# Autodesk Inventor assembly: ASY NDM-VOS_powder_hopper
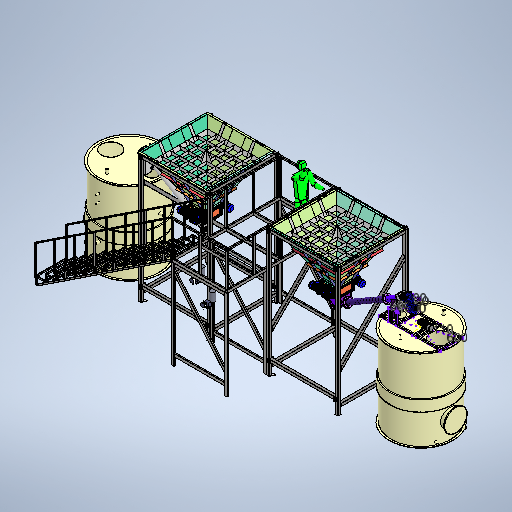
[picture p0: Inventor's stored thumbnail of the model, 512x512]
Saved by Autodesk Inventor 2025 (Build 290162010, 162A)
## iProperties
Created: 2024-07-24
Part Number: ASY NDM-VOS_powder_hopper
Document SubType Name: Assembly
Designer: admin
Author: admin
## Documents named in this file (28)
- C:\Users\pokla\Documents\Inventor\NDM-VOS_powder_hopper\ASY NDM-VOS_powder_hopper.iam
- C:\Users\pokla\Documents\Inventor\NDM-VOS_powder_hopper\human 01\ч ASY human dummy 01.iam
- C:\Users\pokla\Documents\Inventor\NDM-VOS_powder_hopper\NDM-VOS dummy3.ipt
- C:\Users\pokla\Documents\Inventor\NDM-VOS_powder_hopper\NDM-VOS dummy FLOOR.ipt
- C:\Users\pokla\Documents\Inventor\NDM-VOS_powder_hopper\NDM-VOS dummy Crane.ipt
- C:\Users\pokla\Documents\Inventor\NDM-VOS_powder_hopper\NDM-VOS dummy upstairse.ipt
- C:\Users\pokla\Documents\Inventor\NDM-VOS_powder_hopper\Workspaces\Workspace\Cone\ASY MSC 100 cone.iam
- C:\Users\pokla\Documents\Inventor\NDM-VOS_powder_hopper\ASY HPR 200  Frame.iam
- C:\Users\pokla\Documents\Inventor\NDM-VOS_powder_hopper\TM06198C pump.ipt
- C:\Users\pokla\Documents\Inventor\NDM-VOS_powder_hopper\ASY_Ступень.iam
- C:\Users\pokla\Documents\Inventor\NDM-VOS_powder_hopper\ASY стойка.iam
- C:\Users\pokla\Documents\Inventor\NDM-VOS_powder_hopper\ASY NVPH-400 shredder.iam
- C:\Users\admin\YandexDisk-badmisterfox\домашниий пк\Inventor\Content Center Files\en-US\ISO 4775\ISO 4775 - M12.ipt
- C:\Users\pokla\Documents\Inventor\NDM-VOS_powder_hopper\ASY NVPH-300 hopper.iam
- C:\Users\pokla\Documents\Inventor\NDM-VOS_powder_hopper\ASY Augur motor frame 500.iam
- C:\Users\pokla\Documents\Inventor\NDM-VOS_powder_hopper\3d party\motor-reductor NMRV040\motor-reductor NMRV040.iam
- C:\Users\pokla\Documents\Inventor\NDM-VOS_powder_hopper\3d party\Mixer 22.04.24\ASY mixer 3.iam
- C:\Users\pokla\Documents\Inventor\NDM-VOS_powder_hopper\NDM-VOS 777 sredder wall 7.ipt
- C:\Users\pokla\Documents\Inventor\NDM-VOS_powder_hopper\NDM-VOS 778 engine plate.ipt
- C:\Users\pokla\Documents\Inventor\NDM-VOS_powder_hopper\3d party\PCRV071-063SHFA_MS71B5\PCRV071-063SHFA_MS71B5\PCRV071-063SHFA_MS71B5.ipt
- C:\Users\pokla\Documents\Inventor\NDM-VOS_powder_hopper\NDM-VOS 712 flange.ipt
- C:\Users\pokla\Documents\Inventor\NDM-VOS_powder_hopper\NDM-VOS 913 flange bolt.ipt
- C:\Users\pokla\Documents\Inventor\NDM-VOS_powder_hopper\NDM-VOS 715 flange.ipt
- C:\Users\pokla\Documents\Inventor\NDM-VOS_powder_hopper\FL3.6.2  Motor pillar.ipt
- C:\Users\pokla\Documents\Inventor\NDM-VOS_powder_hopper\ASY платформа.iam
- C:\Users\pokla\Documents\Inventor\NDM-VOS_powder_hopper\ISO 4019 - 40x20x2 - 4381,295.ipt
- C:\Users\pokla\Documents\Inventor\NDM-VOS_powder_hopper\ISO 4019 - 40x20x2 - 950.ipt
- C:\Users\pokla\Documents\Inventor\NDM-VOS_powder_hopper\ISO 4019 - 40x20x2 - 3000.ipt
## Components (66 placed, 27 different names)
1. NDM-VOS dummy3:2 — Mate:6, Mate:8, Mate:9
2. ч ASY human dummy 01:1 [sub-assembly]
3. NDM-VOS dummy FLOOR:1 — Mate:5, Mate:6, Mate:8, Mate:10, Mate:18
4. NDM-VOS dummy Crane:1 — Mate:10
5. NDM-VOS dummy upstairse:1 — Mate:18
6. ASY MSC 100 CONE:1 [sub-assembly] — Mate:20, Rigid:27, Mate:35, Mate:36
7. ASY HPR 200  Frame:1 [sub-assembly] — Mate:20, Rigid:31, Rigid:32, Mate:35, Mate:36
8. TM06198C pump:1
9. ASY HPR 200  Frame:2 [sub-assembly] — Rigid:33, Mate:47
10. ASY стойка:1 [sub-assembly] — Rigid:32, Rigid:33, Mate:46, Flush:37
11. ASY стойка:2 [sub-assembly] — Rigid:4, Rigid:31, Mate:37, Flush:29, Flush:30
12. ASY стойка:3 [sub-assembly] — Rigid:4
13. ASY MSC 100 CONE:2 [sub-assembly] — Rigid:29
14. TM06198C pump:2
15. ASY NVPH-400 shredder:1 [sub-assembly] — Rigid:27, Mate:31, Mate:32
16. ISO 4775 M12:1 — Mate:31, Mate:32
17. ASY NVPH-300 hopper:1 [sub-assembly] — Rigid:34
18. ASY NVPH-400 shredder:2 [sub-assembly] — Rigid:29, Rigid:30
19. ASY NVPH-300 hopper:2 [sub-assembly] — Rigid:30
20. NDM-VOS dummy3:1 — Mate:5, Mate:9
21. ASY Augur motor frame 500:1 [sub-assembly] — Mate:40, Mate:42, Flush:34, Mate:43, Flush:35, Mate:44, Mate:45, Flush:36
22. motor-reductor NMRV040:1 [sub-assembly] — Rotational:15
23. ASY mixer 3:1 [sub-assembly] — Rotational:15
24. NDM-VOS 112 sredder wall sub:1 — Rigid:34, Rigid:35
25. NDM-VOS 778 engine plate:1 — Rigid:35, Rigid:36, Mate:39, Mate:41
26. PCRV071-063SHFA_MS71B5:1 — Rigid:36
27. NDM-VOS 712 flange:1 — Mate:39, Mate:40, Flush:32, Flush:33
28. NDM-VOS 913 flange bolt:1 — Mate:37, Flush:29, Flush:30, Rigid:37
29. NDM-VOS 913 flange bolt:2 — Rigid:37
30. NDM-VOS 712 flange:2 — Mate:41, Flush:32, Flush:33
31. NDM-VOS 715 flange:1 — Mate:42, Flush:34
32. FL3.6.2  Motor pillar:1 — Mate:43, Flush:35, Mate:44
33. NDM-VOS 715 flange:2 — Mate:45, Flush:36
34. ASY платформа:1 [sub-assembly] — Mate:46, Flush:37, Mate:47, Mate:48, Mate:49, Flush:38
35. ISO 4019 - 40x20x2 - 4381,295:1 — Rigid:38
36. ISO 4019 - 40x20x2 - 4381,295:2 — Rigid:39
37. ISO 4019 - 40x20x2 - 3000:1 — Rigid:40
38. ISO 4019 - 40x20x2 - 3000:2 — Rigid:41
39. ASY_Ступень:1 [sub-assembly] — Mate:48, Mate:49, Flush:38
40. ASY_Ступень:2 [sub-assembly]
41. ASY_Ступень:3 [sub-assembly]
42. ASY_Ступень:4 [sub-assembly]
43. ASY_Ступень:5 [sub-assembly]
44. ASY_Ступень:6 [sub-assembly]
45. ASY_Ступень:7 [sub-assembly]
46. ASY_Ступень:8 [sub-assembly]
47. ASY_Ступень:9 [sub-assembly]
48. ASY_Ступень:10 [sub-assembly]
49. ASY_Ступень:11 [sub-assembly]
50. ASY_Ступень:12 [sub-assembly]
51. ASY_Ступень:13 [sub-assembly]
52. ASY_Ступень:14 [sub-assembly] — Rigid:38, Rigid:39, Mate:50, Flush:39, Flush:40, Mate:51, Flush:41, Flush:42
53. ISO 4019 - 40x20x2 - 950:1 — Mate:50, Flush:39, Flush:40, Rigid:40
54. ISO 4019 - 40x20x2 - 950:2 — Mate:51, Flush:41, Flush:42, Rigid:41
55. ISO 4019 - 40x20x2 - 950:3
56. ISO 4019 - 40x20x2 - 950:4
57. ISO 4019 - 40x20x2 - 950:5
58. ISO 4019 - 40x20x2 - 950:6
59. ISO 4019 - 40x20x2 - 950:7
60. ISO 4019 - 40x20x2 - 950:8
61. ISO 4019 - 40x20x2 - 950:9
62. ISO 4019 - 40x20x2 - 950:10
63. ISO 4019 - 40x20x2 - 950:11
64. ISO 4019 - 40x20x2 - 950:12
65. ISO 4019 - 40x20x2 - 950:13
66. ISO 4019 - 40x20x2 - 950:14
## Component patterns: (14 elements, first: ASY_Ступень:1), (7 elements, first: ISO 4019 - 40x20x2 - 950:1 + ISO 4019 - 40x20x2 - 950:2)
## Relationships (63: Mate 29, Flush 17, WeldJoint 16, RevoluteJoint 1)
- Mate:5: NDM-VOS dummy FLOOR:1 ↔ NDM-VOS dummy3:1
- Mate:6: NDM-VOS dummy3:2 ↔ NDM-VOS dummy FLOOR:1
- Mate:8 (1200 mm): NDM-VOS dummy3:2 ↔ NDM-VOS dummy FLOOR:1
- Mate:9 (-1830 mm): NDM-VOS dummy3:2 ↔ NDM-VOS dummy3:1
- Mate:10 (3500 mm): NDM-VOS dummy FLOOR:1 ↔ NDM-VOS dummy Crane:1
- [Mate]: NDM-VOS dummy3:2 ↔ ASY MSC 100 CONE:1
- Mate:18: NDM-VOS dummy FLOOR:1 ↔ NDM-VOS dummy upstairse:1
- [Flush]: ASY HPR 200  Frame:1
- Mate:20: ASY MSC 100 CONE:1 ↔ ASY HPR 200  Frame:1
- Rigid:4 [WeldJoint] (1000 mm): ASY стойка:2 ↔ ASY стойка:3
- Rigid:27 [WeldJoint]: ASY MSC 100 CONE:1 ↔ ASY NVPH-400 shredder:1
- [WeldJoint]: ASY NVPH-400 shredder:1 ↔ ASY NVPH-300 hopper:1
- [Mate]: ASY NVPH-400 shredder:1 ↔ ASY NVPH-300 hopper:1
- [Flush]: ASY NVPH-400 shredder:1 ↔ ASY NVPH-300 hopper:1
- Mate:31: ASY NVPH-400 shredder:1 ↔ ISO 4775 M12:1
- Mate:32: ASY NVPH-400 shredder:1 ↔ ISO 4775 M12:1
- [Mate]: ASY NVPH-400 shredder:1 ↔ ASY NVPH-300 hopper:1
- Rigid:29 [WeldJoint]: ASY MSC 100 CONE:2 ↔ ASY NVPH-400 shredder:2
- Rigid:30 [WeldJoint]: ASY NVPH-400 shredder:2 ↔ ASY NVPH-300 hopper:2
- [Flush]: NDM-VOS dummy3:1 ↔ ASY Augur motor frame 500:1
- [Mate]: NDM-VOS dummy3:1 ↔ ASY Augur motor frame 500:1
- [Flush]: NDM-VOS dummy3:1 ↔ ASY Augur motor frame 500:1
- Rigid:31 [WeldJoint]: ASY HPR 200  Frame:1 ↔ ASY стойка:2
- Rigid:32 [WeldJoint]: ASY HPR 200  Frame:1 ↔ ASY стойка:1
- Rigid:33 [WeldJoint]: ASY HPR 200  Frame:2 ↔ ASY стойка:1
- Mate:35: ASY MSC 100 CONE:1 ↔ ASY HPR 200  Frame:1
- Mate:36: ASY MSC 100 CONE:1 ↔ ASY HPR 200  Frame:1
- Rotational:15 [RevoluteJoint]: motor-reductor NMRV040:1 ↔ ASY mixer 3:1
- Mate:37: ASY стойка:2 ↔ NDM-VOS 913 flange bolt:1
- Flush:29: ASY стойка:2 ↔ NDM-VOS 913 flange bolt:1
- Flush:30: ASY стойка:2 ↔ NDM-VOS 913 flange bolt:1
- Rigid:34 [WeldJoint]: ASY NVPH-300 hopper:1 ↔ NDM-VOS 112 sredder wall sub:1
- Rigid:35 [WeldJoint]: NDM-VOS 112 sredder wall sub:1 ↔ NDM-VOS 778 engine plate:1
- Rigid:36 [WeldJoint]: NDM-VOS 778 engine plate:1 ↔ PCRV071-063SHFA_MS71B5:1
- Mate:39: NDM-VOS 778 engine plate:1 ↔ NDM-VOS 712 flange:1
- Mate:40 (380 mm): ASY Augur motor frame 500:1 ↔ NDM-VOS 712 flange:1
- Mate:41: NDM-VOS 778 engine plate:1 ↔ NDM-VOS 712 flange:2
- Flush:32: NDM-VOS 712 flange:1 ↔ NDM-VOS 712 flange:2
- Flush:33: NDM-VOS 712 flange:1 ↔ NDM-VOS 712 flange:2
- Mate:42: ASY Augur motor frame 500:1 ↔ NDM-VOS 715 flange:1
- Flush:34: ASY Augur motor frame 500:1 ↔ NDM-VOS 715 flange:1
- Mate:43: ASY Augur motor frame 500:1 ↔ FL3.6.2  Motor pillar:1
- Flush:35: ASY Augur motor frame 500:1 ↔ FL3.6.2  Motor pillar:1
- Mate:44: ASY Augur motor frame 500:1 ↔ FL3.6.2  Motor pillar:1
- Mate:45: ASY Augur motor frame 500:1 ↔ NDM-VOS 715 flange:2
- Flush:36: ASY Augur motor frame 500:1 ↔ NDM-VOS 715 flange:2
- Rigid:37 [WeldJoint]: NDM-VOS 913 flange bolt:1 ↔ NDM-VOS 913 flange bolt:2
- Mate:46: ASY стойка:1 ↔ ASY платформа:1
- Flush:37: ASY стойка:1 ↔ ASY платформа:1
- Mate:47: ASY HPR 200  Frame:2 ↔ ASY платформа:1
- Mate:48: ASY платформа:1 ↔ ASY_Ступень:1
- Mate:49: ASY платформа:1 ↔ ASY_Ступень:1
- Flush:38: ASY платформа:1 ↔ ASY_Ступень:1
- Rigid:38 [WeldJoint]: ISO 4019 - 40x20x2 - 4381,295:1 ↔ ASY_Ступень:14
- Rigid:39 [WeldJoint]: ISO 4019 - 40x20x2 - 4381,295:2 ↔ ASY_Ступень:14
- Mate:50: ASY_Ступень:14 ↔ ISO 4019 - 40x20x2 - 950:1
- Flush:39 (10 mm): ASY_Ступень:14 ↔ ISO 4019 - 40x20x2 - 950:1
- Flush:40 (5 mm): ASY_Ступень:14 ↔ ISO 4019 - 40x20x2 - 950:1
- Mate:51: ASY_Ступень:14 ↔ ISO 4019 - 40x20x2 - 950:2
- Flush:41 (10 mm): ASY_Ступень:14 ↔ ISO 4019 - 40x20x2 - 950:2
- Flush:42 (5 mm): ASY_Ступень:14 ↔ ISO 4019 - 40x20x2 - 950:2
- Rigid:40 [WeldJoint]: ISO 4019 - 40x20x2 - 3000:1 ↔ ISO 4019 - 40x20x2 - 950:1
- Rigid:41 [WeldJoint]: ISO 4019 - 40x20x2 - 3000:2 ↔ ISO 4019 - 40x20x2 - 950:2
